# Autodesk Inventor assembly: Roller Shaft
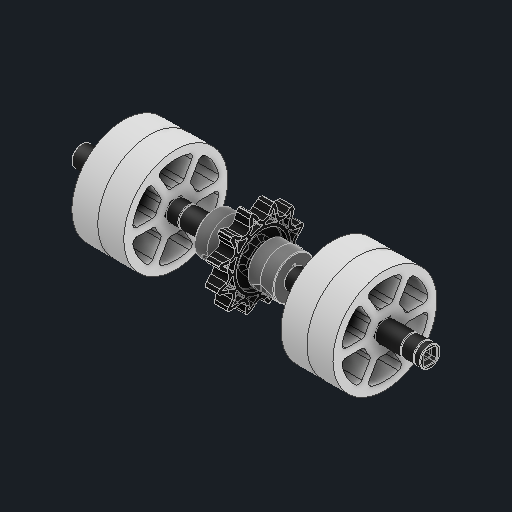
[picture p0: Inventor's stored thumbnail of the model, 512x512]
Saved by Autodesk Inventor 2025 (Build 290162000, 162)
## iProperties
Created: 2024-10-20
Part Number: Roller Shaft
Document SubType Name: Assembly
Designer: Averey Ku
Author: Averey Ku
## Documents named in this file (11)
- D:\VEX\High Stakes\CAD\V2\Hook\Roller Shaft.iam
- D:\VEX\High Stakes\CAD\ROBOPROS-CAD-Inventor\Motion\Sprockets\9P Sprocket\9P 12T Sprocket, No Insert.iam
- D:\VEX\High Stakes\CAD\ROBOPROS-CAD-Inventor\Motion\Sprockets\9P Sprocket.iam
- D:\VEX\High Stakes\CAD\ROBOPROS-CAD-Inventor\Motion\Wheels\Flex Wheels\2.000 Flex Wheel\2.000 30A .500.ipt
- D:\VEX\High Stakes\CAD\ROBOPROS-CAD-Inventor\Motion\Wheels\Flex Wheels\2.000 Flex Wheel.ipt
- D:\VEX\High Stakes\CAD\ROBOPROS-CAD-Inventor\Motion\Shaft HS\HS Shaft Collar.ipt
- D:\VEX\High Stakes\CAD\ROBOPROS-CAD-Inventor\Motion\Shaft HS\HS Spacer\HSpacer .2500.ipt
- D:\VEX\High Stakes\CAD\ROBOPROS-CAD-Inventor\Motion\Shaft HS\HS Spacer.ipt
- D:\VEX\High Stakes\CAD\ROBOPROS-CAD-Inventor\Motion\Shaft HS\HS Spacer\HSpacer .5000.ipt
- D:\VEX\High Stakes\CAD\ROBOPROS-CAD-Inventor\Motion\Shaft HS\HS Spacer\HSpacer .0625.ipt
- D:\VEX\High Stakes\CAD\ROBOPROS-CAD-Inventor\Motion\Shaft HS\HS Spacer\HSpacer .1250.ipt
## Components (17 placed, 7 different names)
1. 9P 12T Sprocket, No Insert:1 [sub-assembly]
2. 2.000 30A .500:1 — Insert:19
3. 2.000 30A .500:2 — Insert:20
4. 2.000 30A .500:3 — Insert:16
5. 2.000 30A .500:4 — Insert:22
6. HS Shaft Collar:1 — Mate:2
7. HSpacer .2500:1 — Insert:18, Insert:19
8. HSpacer .5000:2 — Mate:3, Mate:4, Insert:18
9. HS Shaft Collar:2
10. HSpacer .2500:4 — Insert:22, Insert:23
11. HSpacer .5000:5 — Insert:23
12. HSpacer .0625:7 — Insert:13, Insert:24
13. HSpacer .2500:8 — Insert:13, Insert:16
14. HSpacer .2500:10 — Insert:17, Insert:21
15. HSpacer .1250:11 — Insert:17
16. HSpacer .5000:12 — Insert:20, Insert:21
17. HSpacer .5000:13 — Insert:24
## Relationships (20: Insert 16, Mate 4)
- [Insert]: 2.000 30A .500:1 ↔ 2.000 30A .500:2
- [Insert]: 2.000 30A .500:3 ↔ 2.000 30A .500:4
- [Mate]: 9P 12T Sprocket, No Insert:1 ↔ 2.000 30A .500:1
- [Insert]: 9P 12T Sprocket, No Insert:1 ↔ HS Shaft Collar:1
- [Insert]: HS Shaft Collar:1 ↔ HSpacer .5000:2
- [Insert]: HS Shaft Collar:2 ↔ HSpacer .5000:5
- [Insert]: 9P 12T Sprocket, No Insert:1 ↔ HS Shaft Collar:2
- Mate:2 (6.35 mm): HS Shaft Collar:1
- Mate:3: HSpacer .5000:2
- Mate:4: HSpacer .5000:2
- Insert:13: HSpacer .0625:7 ↔ HSpacer .2500:8
- Insert:16: 2.000 30A .500:3 ↔ HSpacer .2500:8
- Insert:17: HSpacer .2500:10 ↔ HSpacer .1250:11
- Insert:18: HSpacer .2500:1 ↔ HSpacer .5000:2
- Insert:19: 2.000 30A .500:1 ↔ HSpacer .2500:1
- Insert:20: 2.000 30A .500:2 ↔ HSpacer .5000:12
- Insert:21: HSpacer .2500:10 ↔ HSpacer .5000:12
- Insert:22: 2.000 30A .500:4 ↔ HSpacer .2500:4
- Insert:23: HSpacer .2500:4 ↔ HSpacer .5000:5
- Insert:24: HSpacer .0625:7 ↔ HSpacer .5000:13
## Named parameters: d61_d58 = 0 mm, d42_d40 = 0 mm
